# Autodesk Inventor assembly: Right-Brush
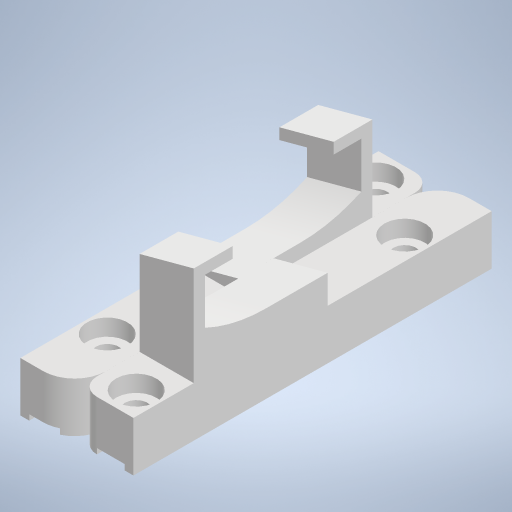
[picture p0: Inventor's stored thumbnail of the model, 512x512]
Saved by Autodesk Inventor 2024 (Build 280153000, 153)
## iProperties
Created: 2023-12-13
Part Number: Right-Brush
Document SubType Name: Assembly
Designer: shaun
Author: shaun
## Documents named in this file (3)
- Z:\VirtualBox VMs\Baxter\ROS2-Baxter\3D Models\Gripper V1\Right-Brush.iam
- Z:\VirtualBox VMs\Baxter\ROS2-Baxter\3D Models\Gripper V1\Right-Brush-Bottom.ipt
- Z:\VirtualBox VMs\Baxter\ROS2-Baxter\3D Models\Gripper V1\Right-Brush-Top.ipt
## Components (2 placed, 2 different names)
1. Right-Brush-Bottom:1 — Flush:1, Mate:1
2. Right-Brush-Top:1 — Flush:1, Mate:1, Mate:2
## Relationships (3: Mate 2, Flush 1)
- Flush:1: Right-Brush-Bottom:1 ↔ Right-Brush-Top:1
- Mate:1: Right-Brush-Bottom:1 ↔ Right-Brush-Top:1
- Mate:2: Right-Brush-Top:1
